# Autodesk Inventor assembly: canaletaLateral
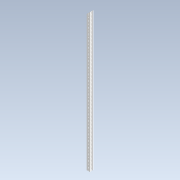
[picture p0: Inventor's stored thumbnail of the model, 180x180]
Saved by Autodesk Inventor 2021 (Build 250183000, 183)
## iProperties
Created: 2021-08-23
Part Number: canaletaLateral
Document SubType Name: Assembly
Designer: Andrés Holguín
Author: Andrés Holguín
## Documents named in this file (2)
- C:\Users\andre\Documents\GitHub\Dis.-Mecatronico-E6\inventor proyecto\Tablero\Canaletas\canaletaLateral.iam
- C:\Users\andre\Documents\GitHub\Dis.-Mecatronico-E6\inventor proyecto\Tablero\Canaletas\7308-1.iam
## Components (12 placed, 1 different names)
1. 7308-1:2 [sub-assembly]
2. 7308-1:3 [sub-assembly]
3. 7308-1:4 [sub-assembly]
4. 7308-1:5 [sub-assembly]
5. 7308-1:6 [sub-assembly]
6. 7308-1:7 [sub-assembly]
7. 7308-1:8 [sub-assembly]
8. 7308-1:9 [sub-assembly]
9. 7308-1:10 [sub-assembly]
10. 7308-1:11 [sub-assembly]
11. 7308-1:12 [sub-assembly]
12. 7308-1:13 [sub-assembly] — Mate:1, Angle:1
## Relationships (13: WeldJoint 11, Mate 1, Angle 1)
- [WeldJoint]: 7308-1:2 ↔ 7308-1:4
- [WeldJoint]: 7308-1:4 ↔ 7308-1:5
- [WeldJoint]: 7308-1:6 ↔ 7308-1:8
- [WeldJoint]: 7308-1:3 ↔ 7308-1:6
- [WeldJoint]: 7308-1:3 ↔ 7308-1:7
- [WeldJoint]: 7308-1:5 ↔ 7308-1:9
- [WeldJoint]: 7308-1:8 ↔ 7308-1:9
- [WeldJoint]: 7308-1:11 ↔ 7308-1:12
- [WeldJoint]: 7308-1:10 ↔ 7308-1:12
- [WeldJoint]: 7308-1:7 ↔ 7308-1:10
- [WeldJoint]: 7308-1:11 ↔ 7308-1:13
- Mate:1: 7308-1:13
- Angle:1 (-45 deg): 7308-1:13
